# Autodesk Inventor assembly: 全体v1
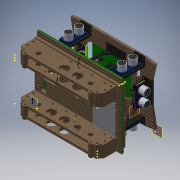
[picture p0: Inventor's stored thumbnail of the model, 180x180]
Saved by Autodesk Inventor 2018 (Build 220112000, 112)
## iProperties
Created: 2018-11-27
Part Number: 全体v1
Material: 一般
Document SubType Name: Assembly
Designer: shun2
Author: shun2
## Documents named in this file (17)
- C:\Users\shun2\OneDrive\おそらく最新版(2018.7.31)\全体v1.iam
- C:\Users\shun2\OneDrive\おそらく最新版(2018.7.31)\ギアボックス\ギアボックスv2.iam
- C:\Users\shun2\OneDrive\おそらく最新版(2018.7.31)\1枚目\一枚目.ipt
- C:\Users\shun2\OneDrive\おそらく最新版(2018.7.31)\基板保護2018.8.7.ipt
- C:\Users\shun2\OneDrive\おそらく最新版(2018.7.31)\2枚目\2枚目.ipt
- C:\Users\shun2\OneDrive\おそらく最新版(2018.7.31)\ステッピング固定具.ipt
- C:\Users\shun2\OneDrive\おそらく最新版(2018.7.31)\レスキューキット投下機構.ipt
- C:\Users\shun2\OneDrive\おそらく最新版(2018.7.31)\レスキューキット接続.ipt
- C:\Users\shun2\OneDrive\おそらく最新版(2018.7.31)\3枚目\3枚目v4.ipt
- C:\Users\shun2\OneDrive\おそらく最新版(2018.7.31)\ping-module.iam
- C:\Users\shun2\OneDrive\おそらく最新版(2018.7.31)\pingmodule-y.iam
- C:\Users\shun2\OneDrive\おそらく最新版(2018.7.31)\OpenMV&Ping.iam
- C:\Users\shun2\OneDrive\おそらく最新版(2018.7.31)\OpenMVMount-Tate.iam
- C:\Users\shun2\OneDrive\おそらく最新版(2018.7.31)\Color.ipt
- C:\Users\shun2\OneDrive\おそらく最新版(2018.7.31)\モタドラ.ipt
- C:\Users\shun2\OneDrive\おそらく最新版(2018.7.31)\メイン基板.ipt
- C:\Users\shun2\OneDrive\おそらく最新版(2018.7.31)\Aquila-2018-Under.ipt
## Components (21 placed, 16 different names)
1. ギアボックスv2:1 [sub-assembly] — メイト:1, フラッシュ:2, フラッシュ:3
2. ギアボックスv2:2 [sub-assembly] — メイト:2, フラッシュ:1, フラッシュ:4
3. 一枚目:1 — メイト:1, メイト:2, フラッシュ:1, フラッシュ:2, フラッシュ:3, フラッシュ:4, メイト:3, メイト:4, メイト:5, メイト:44, メイト:45, メイト:46, メイト:47, メイト:48, メイト:49, メイト:53, メイト:54, メイト:55
4. 基板保護2018.8.7:1 — メイト:3, メイト:4, メイト:5, メイト:6, メイト:7, メイト:8
5. 2枚目:1 — メイト:6, メイト:7, メイト:8, メイト:9, メイト:10, メイト:11, メイト:15, メイト:41, メイト:42, メイト:43
6. ステッピング固定具:2 — メイト:9, メイト:10, メイト:11, 回転:1
7. レスキューキット投下機構:1 — メイト:12, メイト:13, メイト:14, メイト:15
8. レスキューキット接続:1 — メイト:12, メイト:13, メイト:14, 回転:1
9. 3枚目v4:1 — メイト:16, メイト:17, メイト:18, メイト:19, メイト:20, メイト:21, メイト:23, メイト:24, メイト:25, メイト:26, メイト:27, メイト:28, メイト:29, メイト:30, メイト:31, メイト:32, メイト:33, メイト:34, メイト:35, メイト:36, メイト:37, メイト:38, メイト:39, メイト:40, メイト:41, メイト:42, メイト:43, メイト:50, メイト:51, メイト:52
10. ping-module:1 [sub-assembly] — メイト:16, メイト:17, メイト:18
11. ping-module:2 [sub-assembly] — メイト:19, メイト:20, メイト:21
12. ping-module:3 [sub-assembly] — メイト:23, メイト:24, メイト:25
13. ping-module:4 [sub-assembly] — メイト:26, メイト:27, メイト:28
14. pingmodule-y:1 [sub-assembly] — メイト:29, メイト:30, メイト:31
15. OpenMV&Ping:1 [sub-assembly] — メイト:32, メイト:33, メイト:34
16. OpenMVMount-Tate:1 [sub-assembly] — メイト:38, メイト:39, メイト:40
17. OpenMVMount-Tate:2 [sub-assembly] — メイト:35, メイト:36, メイト:37
18. Color:1 — メイト:44, メイト:45, メイト:46
19. モタドラ:1 — メイト:47, メイト:48, メイト:49
20. メイン基板:1 — メイト:50, メイト:51, メイト:52
21. Aquila-2018-Under:2 — メイト:53, メイト:54, メイト:55
## Relationships (59: Mate 54, Flush 4, RevoluteJoint 1)
- メイト:1 [Mate] (3 mm): ギアボックスv2:1 ↔ 一枚目:1
- メイト:2 [Mate] (3 mm): ギアボックスv2:2 ↔ 一枚目:1
- フラッシュ:1 [Flush]: ギアボックスv2:2 ↔ 一枚目:1
- フラッシュ:2 [Flush]: ギアボックスv2:1 ↔ 一枚目:1
- フラッシュ:3 [Flush] (2 mm): ギアボックスv2:1 ↔ 一枚目:1
- フラッシュ:4 [Flush] (2 mm): ギアボックスv2:2 ↔ 一枚目:1
- メイト:3 [Mate] (0.2 mm): 一枚目:1 ↔ 基板保護2018.8.7:1
- メイト:4 [Mate]: 一枚目:1 ↔ 基板保護2018.8.7:1
- メイト:5 [Mate]: 一枚目:1 ↔ 基板保護2018.8.7:1
- メイト:6 [Mate] (3 mm): 基板保護2018.8.7:1 ↔ 2枚目:1
- メイト:7 [Mate]: 基板保護2018.8.7:1 ↔ 2枚目:1
- メイト:8 [Mate]: 基板保護2018.8.7:1 ↔ 2枚目:1
- メイト:9 [Mate] (12 mm): 2枚目:1 ↔ ステッピング固定具:2
- メイト:10 [Mate]: 2枚目:1 ↔ ステッピング固定具:2
- メイト:11 [Mate]: 2枚目:1 ↔ ステッピング固定具:2
- メイト:12 [Mate]: レスキューキット投下機構:1 ↔ レスキューキット接続:1
- メイト:13 [Mate]: レスキューキット投下機構:1 ↔ レスキューキット接続:1
- メイト:14 [Mate]: レスキューキット投下機構:1 ↔ レスキューキット接続:1
- メイト:15 [Mate] (3 mm): 2枚目:1 ↔ レスキューキット投下機構:1
- 回転:1 [RevoluteJoint] (3.5 mm): ステッピング固定具:2 ↔ レスキューキット接続:1
- メイト:16 [Mate]: 3枚目v4:1 ↔ ping-module:1
- メイト:17 [Mate]: 3枚目v4:1 ↔ ping-module:1
- メイト:18 [Mate]: 3枚目v4:1 ↔ ping-module:1
- メイト:19 [Mate]: 3枚目v4:1 ↔ ping-module:2
- メイト:20 [Mate]: 3枚目v4:1 ↔ ping-module:2
- メイト:21 [Mate]: 3枚目v4:1 ↔ ping-module:2
- メイト:23 [Mate]: 3枚目v4:1 ↔ ping-module:3
- メイト:24 [Mate]: 3枚目v4:1 ↔ ping-module:3
- メイト:25 [Mate]: 3枚目v4:1 ↔ ping-module:3
- メイト:26 [Mate]: 3枚目v4:1 ↔ ping-module:4
- メイト:27 [Mate]: 3枚目v4:1 ↔ ping-module:4
- メイト:28 [Mate]: 3枚目v4:1 ↔ ping-module:4
- メイト:29 [Mate]: 3枚目v4:1 ↔ pingmodule-y:1
- メイト:30 [Mate]: 3枚目v4:1 ↔ pingmodule-y:1
- メイト:31 [Mate]: 3枚目v4:1 ↔ pingmodule-y:1
- メイト:32 [Mate]: 3枚目v4:1 ↔ OpenMV&Ping:1
- メイト:33 [Mate]: 3枚目v4:1 ↔ OpenMV&Ping:1
- メイト:34 [Mate]: 3枚目v4:1 ↔ OpenMV&Ping:1
- メイト:35 [Mate]: 3枚目v4:1 ↔ OpenMVMount-Tate:2
- メイト:36 [Mate]: 3枚目v4:1 ↔ OpenMVMount-Tate:2
- メイト:37 [Mate]: 3枚目v4:1 ↔ OpenMVMount-Tate:2
- メイト:38 [Mate]: 3枚目v4:1 ↔ OpenMVMount-Tate:1
- メイト:39 [Mate]: 3枚目v4:1 ↔ OpenMVMount-Tate:1
- メイト:40 [Mate]: 3枚目v4:1 ↔ OpenMVMount-Tate:1
- メイト:41 [Mate] (68 mm): 2枚目:1 ↔ 3枚目v4:1
- メイト:42 [Mate]: 2枚目:1 ↔ 3枚目v4:1
- メイト:43 [Mate]: 2枚目:1 ↔ 3枚目v4:1
- メイト:44 [Mate] (40 mm): 一枚目:1 ↔ Color:1
- メイト:45 [Mate]: 一枚目:1 ↔ Color:1
- メイト:46 [Mate]: 一枚目:1 ↔ Color:1
- メイト:47 [Mate] (8 mm): 一枚目:1 ↔ モタドラ:1
- メイト:48 [Mate]: 一枚目:1 ↔ モタドラ:1
- メイト:49 [Mate]: 一枚目:1 ↔ モタドラ:1
- メイト:50 [Mate] (8 mm): 3枚目v4:1 ↔ メイン基板:1
- メイト:51 [Mate]: 3枚目v4:1 ↔ メイン基板:1
- メイト:52 [Mate]: 3枚目v4:1 ↔ メイン基板:1
- メイト:53 [Mate] (3 mm): 一枚目:1 ↔ Aquila-2018-Under:2
- メイト:54 [Mate]: 一枚目:1 ↔ Aquila-2018-Under:2
- メイト:55 [Mate]: 一枚目:1 ↔ Aquila-2018-Under:2
